# Autodesk Inventor assembly: Axel_genom_ifylld_PIP-KIL_02
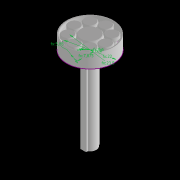
[picture p0: Inventor's stored thumbnail of the model, 180x180]
Saved by Autodesk Inventor 2020 (Build 240168000, 168)
## iProperties
Created: 2020-11-21
Part Number: Axel_genom_ifylld_PIP-KIL_02
Document SubType Name: Assembly
Designer: Gottfrid
Author: Gottfrid
## Documents named in this file (3)
- D:\PROJEKT\GENERATOR V.1\3D-filer [2020-11-21]\Axel_genom_ifylld_PIP-KIL_02.iam
- D:\PROJEKT\GENERATOR V.1\3D-filer [2020-11-21]\Axel_parametriserad_02.ipt
- D:\PROJEKT\GENERATOR V.1\3D-filer [2020-11-21]\PIP-KL_parametriserad_02_testarFyllai.ipt
## Components (2 placed, 2 different names)
1. Axel_parametriserad_02:1 — Mate:1, Mate:2
2. PIP-KL_parametriserad_02_testarFyllai:1 — Mate:1, Mate:2
## Relationships (2: Mate 2)
- Mate:1: Axel_parametriserad_02:1 ↔ PIP-KL_parametriserad_02_testarFyllai:1
- Mate:2: Axel_parametriserad_02:1 ↔ PIP-KL_parametriserad_02_testarFyllai:1
